# Autodesk Inventor assembly: X rail L + dual mount b
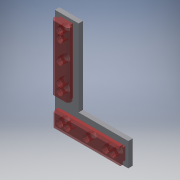
[picture p0: Inventor's stored thumbnail of the model, 180x180]
Saved by Autodesk Inventor 2018 (Build 220112000, 112)
## iProperties
Created: 2017-11-11
Part Number: X rail L + dual mount b
Document SubType Name: Assembly
Designer: ball
Author: ball
## Documents named in this file (3)
- C:\FTC\2017Robot\X rail L + dual mount b.iam
- C:\FTC\Actobotics\585 parts\585076.ipt
- C:\FTC\Actobotics\585 parts\585718.ipt
## Components (3 placed, 2 different names)
1. 585076:1 — Mate:1, Mate:2, Mate:3, Mate:4, Mate:5, Mate:6
2. 585718:1 — Mate:1, Mate:2, Mate:3
3. 585718:2 — Mate:4, Mate:5, Mate:6
## Relationships (6: Mate 6)
- Mate:1: 585076:1 ↔ 585718:1
- Mate:2: 585076:1 ↔ 585718:1
- Mate:3: 585076:1 ↔ 585718:1
- Mate:4: 585076:1 ↔ 585718:2
- Mate:5: 585076:1 ↔ 585718:2
- Mate:6: 585076:1 ↔ 585718:2
